# Autodesk Inventor assembly: Lidar Sensor Lexan Assembly
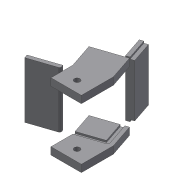
[picture p0: Inventor's stored thumbnail of the model, 180x180]
Saved by Autodesk Inventor 2018.3 (Build 223284000, 284)
## iProperties
Created: 2019-02-26
Part Number: Lidar Sensor Lexan Assembly
Document SubType Name: Assembly
Designer: aye06091
Mass: 24.6528 g
Surface Area: 127.634 cm^2
Volume: 24.6528 cm^3
Density: 1 g/cm^3
Author: aye06091
## Documents named in this file (5)
- Y:\DeSimony-R\Senior R&D\4 R&D Shared Folder\VisiStick\VisiStick (Inventor)\Physical Parts\Lidar Sensor Lexan Assembly.iam
- Y:\DeSimony-R\Senior R&D\4 R&D Shared Folder\VisiStick\VisiStick (Inventor)\Physical Parts\Lidar Sensor CAse Piece 1.ipt
- Y:\DeSimony-R\Senior R&D\4 R&D Shared Folder\VisiStick\VisiStick (Inventor)\Physical Parts\Lidar Sensor Case Piece 2.ipt
- Y:\DeSimony-R\Senior R&D\4 R&D Shared Folder\VisiStick\VisiStick (Inventor)\Physical Parts\Lidar Sensor Case Piece 3.ipt
- Y:\DeSimony-R\Senior R&D\4 R&D Shared Folder\VisiStick\VisiStick (Inventor)\Physical Parts\Lidar Sensor Case Piece 4.ipt
## Components (4 placed, 4 different names)
1. Lidar Sensor CAse Piece 1:1 — Flush:2, Flush:3, Mate:5, Flush:4, Flush:5
2. Lidar Sensor Case Piece 2:1 — Flush:2, Flush:3, Mate:3, Mate:4, Mate:6, Flush:4, Flush:5
3. Lidar Sensor Case Piece 4:1 — Mate:3, Mate:4
4. Lidar Sensor Case Piece 3:1 — Mate:5, Mate:6
## Relationships (8: Flush 4, Mate 4)
- Flush:2: Lidar Sensor CAse Piece 1:1 ↔ Lidar Sensor Case Piece 2:1
- Flush:3: Lidar Sensor CAse Piece 1:1 ↔ Lidar Sensor Case Piece 2:1
- Mate:3: Lidar Sensor Case Piece 2:1 ↔ Lidar Sensor Case Piece 4:1
- Mate:4: Lidar Sensor Case Piece 2:1 ↔ Lidar Sensor Case Piece 4:1
- Mate:5: Lidar Sensor CAse Piece 1:1 ↔ Lidar Sensor Case Piece 3:1
- Mate:6: Lidar Sensor Case Piece 2:1 ↔ Lidar Sensor Case Piece 3:1
- Flush:4: Lidar Sensor CAse Piece 1:1 ↔ Lidar Sensor Case Piece 2:1
- Flush:5: Lidar Sensor CAse Piece 1:1 ↔ Lidar Sensor Case Piece 2:1
